# Autodesk Inventor assembly: EsagonoScreeenChiuso
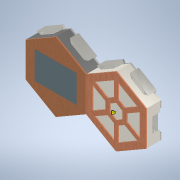
[picture p0: Inventor's stored thumbnail of the model, 180x180]
Saved by Autodesk Inventor 2020 (Build 240168000, 168)
## iProperties
Created: 2020-04-22
Part Number: EsagonoScreeenChiuso
Document SubType Name: Assembly
Designer: Samuele
Author: Samuele
## Documents named in this file (7)
- C:\EsagoniMalsani\ModelliComponenti\EsagonoScreeenChiuso.iam
- C:\EsagoniMalsani\ModelliComponenti\Esagoni\HexagoneBack.ipt
- C:\EsagoniMalsani\ModelliComponenti\Componenti\TouchLCD.ipt
- C:\EsagoniMalsani\ModelliComponenti\Esagoni\ScreenFrontalino.ipt
- C:\EsagoniMalsani\ModelliComponenti\Esagoni\ScreenModule.ipt
- C:\EsagoniMalsani\ModelliComponenti\Esagoni\LightModule.ipt
- C:\EsagoniMalsani\ModelliComponenti\Esagoni\LightFrontalino.ipt
## Components (7 placed, 6 different names)
1. ScreenModule:1 — Flush:1, Mate:1, Flush:2, Flush:4, Flush:5, Mate:4, Flush:10, Mate:8, Mate:9
2. TouchLCD:1 — Mate:2, Mate:3, Flush:3
3. HexagoneBack:1 — Flush:4, Flush:5, Mate:4
4. ScreenFrontalino:1 — Flush:1, Mate:1, Flush:2, Mate:2, Mate:3, Flush:3
5. LightModule:1 — Mate:5, Flush:6, Flush:7, Flush:8, Flush:9, Mate:7, Flush:10, Mate:8, Mate:9
6. LightFrontalino:1 — Mate:5, Flush:6, Flush:7
7. HexagoneBack:2 — Flush:8, Flush:9, Mate:7
## Relationships (18: Flush 10, Mate 8)
- Flush:1: ScreenModule:1 ↔ ScreenFrontalino:1
- Mate:1: ScreenModule:1 ↔ ScreenFrontalino:1
- Flush:2: ScreenModule:1 ↔ ScreenFrontalino:1
- Mate:2: TouchLCD:1 ↔ ScreenFrontalino:1
- Mate:3: TouchLCD:1 ↔ ScreenFrontalino:1
- Flush:3: TouchLCD:1 ↔ ScreenFrontalino:1
- Flush:4: ScreenModule:1 ↔ HexagoneBack:1
- Flush:5: ScreenModule:1 ↔ HexagoneBack:1
- Mate:4: ScreenModule:1 ↔ HexagoneBack:1
- Mate:5: LightModule:1 ↔ LightFrontalino:1
- Flush:6: LightModule:1 ↔ LightFrontalino:1
- Flush:7: LightModule:1 ↔ LightFrontalino:1
- Flush:8: LightModule:1 ↔ HexagoneBack:2
- Flush:9: LightModule:1 ↔ HexagoneBack:2
- Mate:7: LightModule:1 ↔ HexagoneBack:2
- Flush:10: ScreenModule:1 ↔ LightModule:1
- Mate:8: ScreenModule:1 ↔ LightModule:1
- Mate:9: ScreenModule:1 ↔ LightModule:1
